# Autodesk Inventor assembly: Verbindungskabel_seitlich
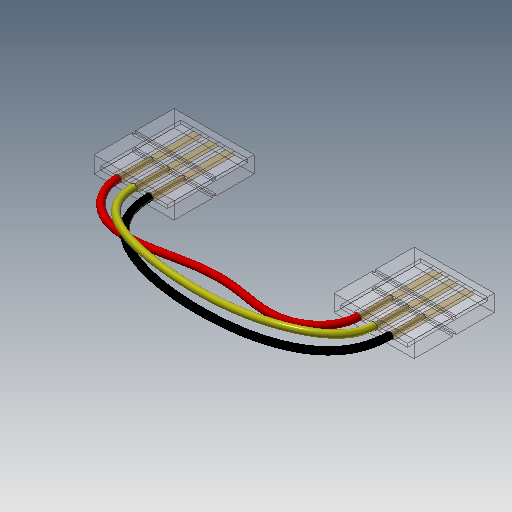
[picture p0: Inventor's stored thumbnail of the model, 512x512]
Saved by Autodesk Inventor 2021.3 (Build 253353000, 353)
## iProperties
Company: Schneeberger Lineartechnik AG
RuleStatus: InUse
Created: 2021-09-28
Part Number: Verbindungskabel_seitlich
User Status: Schnelländerung
Document SubType Name: Assembly
Designer: SRORF
Mass: 0.786999 g
Surface Area: 17.9462 cm^2
Volume: 0.704007 cm^3
Density: 1.11789 g/cm^3
Status: Produktion Freigegeben
ROT_Density: 0.0
PDB_Ident_Ver: =<PDB_Ident> <PDB_Version>
ROT_Weight: 0.001 kg
ROT_Weight_Num: 0.0007869990087500127
Author: SRORF
## Documents named in this file (3)
- C:\kt\WorkSpace\Uhr\CAD\Verbindungskabel_seitlich.iam
- C:\kt\WorkSpace\Uhr\CAD\3_Pin_LED_Verbinder.ipt
- C:\kt\WorkSpace\Uhr\CAD\Verbindungskabel_1.ipt
## Components (3 placed, 2 different names)
1. Verbindungskabel_1:1 — Passend:1, Passend:2, Fluchtend:1
2. 3_Pin_LED_Verbinder:1 — Passend:2
3. 3_Pin_LED_Verbinder:2
## Component patterns: (2 elements, first: 3_Pin_LED_Verbinder:1)
## Relationships (3: Mate 2, Flush 1)
- Passend:1 [Mate]: Verbindungskabel_1:1
- Passend:2 [Mate]: Verbindungskabel_1:1 ↔ 3_Pin_LED_Verbinder:1
- Fluchtend:1 [Flush]: Verbindungskabel_1:1
